# Autodesk Inventor assembly: RollingSquareC1
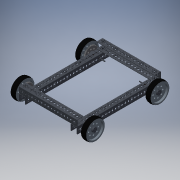
[picture p0: Inventor's stored thumbnail of the model, 180x180]
Saved by Autodesk Inventor 2016 (Build 200138000, 138)
## iProperties
Created: 2015-08-30
Part Number: RollingSquareC1
Document SubType Name: Assembly
Designer: Tim
Author: Tim
## Documents named in this file (7)
- C:\Users\Tim\Documents\GitHub\phi_robotics\3d-models\FTC_Tetrix_KOP_Block_Party\RollingSquareC1.iam
- C:\Users\Tim\Documents\GitHub\phi_robotics\3d-models\FTC_Tetrix_KOP_Block_Party\Tetrix_Kit_FTC\Autodesk Inventor Files\tetrix_c_channel-5.ipt
- C:\Users\Tim\Documents\GitHub\phi_robotics\3d-models\FTC_Tetrix_KOP_Block_Party\Tetrix_Kit_FTC\Autodesk Inventor Files\tetrix_c_channel-4.ipt
- C:\Users\Tim\Documents\GitHub\phi_robotics\3d-models\FTC_Tetrix_KOP_Block_Party\Tetrix_Kit_FTC\Autodesk Inventor Files\tetrix_bushing.ipt
- C:\Users\Tim\Documents\GitHub\phi_robotics\3d-models\FTC_Tetrix_KOP_Block_Party\Tetrix_Kit_FTC\Autodesk Inventor Files\tetrix_axle.ipt
- C:\Users\Tim\Documents\GitHub\phi_robotics\3d-models\FTC_Tetrix_KOP_Block_Party\Tetrix_Kit_FTC\Autodesk Inventor Files\tetrix_739092_2012.iam
- C:\Users\Tim\Documents\GitHub\phi_robotics\3d-models\FTC_Tetrix_KOP_Block_Party\WheelNGear.iam
## Components (24 placed, 6 different names)
1. tetrix_c_channel-5:1 — Mate:1, Mate:3, Rotational:3, Rotational:4, Rotational:6, Rotational:7
2. tetrix_c_channel-5:2 — Mate:2, Mate:4, Rotational:1, Rotational:2, Rotational:11, Rotational:12
3. tetrix_c_channel-4:1 — Mate:1, Mate:2
4. tetrix_c_channel-4:2 — Mate:3, Mate:4
5. tetrix_bushing:1 — Rotational:2
6. tetrix_bushing:2 — Rotational:1, Rotational:9
7. tetrix_bushing:3 — Rotational:3
8. tetrix_bushing:4 — Rotational:4, Rotational:5
9. tetrix_axle:1 — Rotational:5, Rigid:1, Rigid:7
10. tetrix_739092_2012:1 [sub-assembly] — Rigid:1
11. tetrix_bushing:5 — Rotational:6
12. tetrix_bushing:6 — Rotational:7, Rotational:8
13. tetrix_axle:2 — Rigid:2, Rotational:8, Rigid:6
14. tetrix_739092_2012:2 [sub-assembly] — Rigid:2
15. tetrix_axle:3 — Rotational:9, Rigid:3, Rigid:8
16. tetrix_739092_2012:3 [sub-assembly] — Rigid:3
17. tetrix_bushing:7 — Rotational:11
18. tetrix_bushing:8 — Rotational:12, Rotational:13
19. tetrix_axle:4 — Rotational:13, Rigid:4, Rigid:5
20. tetrix_739092_2012:4 [sub-assembly] — Rigid:4
21. WheelNGear:1 [sub-assembly] — Rigid:5
22. WheelNGear:2 [sub-assembly] — Rigid:8
23. WheelNGear:3 [sub-assembly] — Rigid:7
24. WheelNGear:4 [sub-assembly] — Rigid:6
## Relationships (24: RevoluteJoint 12, WeldJoint 8, Mate 4)
- Mate:1: tetrix_c_channel-5:1 ↔ tetrix_c_channel-4:1
- Mate:2: tetrix_c_channel-5:2 ↔ tetrix_c_channel-4:1
- Mate:3: tetrix_c_channel-5:1 ↔ tetrix_c_channel-4:2
- Mate:4: tetrix_c_channel-5:2 ↔ tetrix_c_channel-4:2
- Rotational:1 [RevoluteJoint]: tetrix_c_channel-5:2 ↔ tetrix_bushing:2
- Rotational:2 [RevoluteJoint]: tetrix_c_channel-5:2 ↔ tetrix_bushing:1
- Rotational:3 [RevoluteJoint]: tetrix_c_channel-5:1 ↔ tetrix_bushing:3
- Rotational:4 [RevoluteJoint]: tetrix_c_channel-5:1 ↔ tetrix_bushing:4
- Rotational:5 [RevoluteJoint] (-25 mm): tetrix_bushing:4 ↔ tetrix_axle:1
- Rigid:1 [WeldJoint] (-19.2 mm): tetrix_axle:1 ↔ tetrix_739092_2012:1
- Rotational:6 [RevoluteJoint]: tetrix_c_channel-5:1 ↔ tetrix_bushing:5
- Rotational:7 [RevoluteJoint]: tetrix_c_channel-5:1 ↔ tetrix_bushing:6
- Rigid:2 [WeldJoint] (-19.2 mm): tetrix_axle:2 ↔ tetrix_739092_2012:2
- Rotational:8 [RevoluteJoint] (25 mm): tetrix_bushing:6 ↔ tetrix_axle:2
- Rotational:9 [RevoluteJoint] (25 mm): tetrix_bushing:2 ↔ tetrix_axle:3
- Rigid:3 [WeldJoint] (-19.2 mm): tetrix_axle:3 ↔ tetrix_739092_2012:3
- Rotational:11 [RevoluteJoint]: tetrix_c_channel-5:2 ↔ tetrix_bushing:7
- Rotational:12 [RevoluteJoint]: tetrix_c_channel-5:2 ↔ tetrix_bushing:8
- Rotational:13 [RevoluteJoint] (-25 mm): tetrix_bushing:8 ↔ tetrix_axle:4
- Rigid:4 [WeldJoint] (-19.2 mm): tetrix_axle:4 ↔ tetrix_739092_2012:4
- Rigid:5 [WeldJoint] (-1 mm): tetrix_axle:4 ↔ WheelNGear:1
- Rigid:6 [WeldJoint] (-1 mm): tetrix_axle:2 ↔ WheelNGear:4
- Rigid:7 [WeldJoint] (-1 mm): tetrix_axle:1 ↔ WheelNGear:3
- Rigid:8 [WeldJoint] (-1 mm): tetrix_axle:3 ↔ WheelNGear:2
## Named parameters: d21_d16 = -19.2 mm
